# Autodesk Inventor assembly: Beam
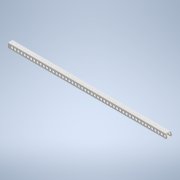
[picture p0: Inventor's stored thumbnail of the model, 180x180]
Saved by Autodesk Inventor 2022 (Build 260153000, 153)
## iProperties
Created: 2022-04-09
Part Number: Beam
Document SubType Name: Weldment
Designer: Patrick
Weld Material: Welded Aluminum-6061
Author: Patrick
## Documents named in this file (2)
- H:\OneDrive - Syddansk Universitet\2. Semester Master\Mekaniske Elementer\Mini Project\Beam.iam
- H:\OneDrive - Syddansk Universitet\2. Semester Master\Mekaniske Elementer\Mini Project\HalfBeam.ipt
## Components (2 placed, 1 different names)
1. HalfBeam:1 — Rigid:1
2. HalfBeam:2 — Rigid:1
## Relationships (1: WeldJoint 1)
- Rigid:1 [WeldJoint]: HalfBeam:1 ↔ HalfBeam:2
